# Autodesk Inventor assembly: endAssembly
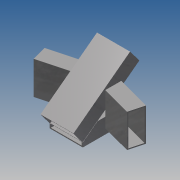
[picture p0: Inventor's stored thumbnail of the model, 180x180]
Saved by Autodesk Inventor 2013 SP2 (Build 170200200, 200)
## iProperties
Created: 2013-12-03
Part Number: endAssembly
Document SubType Name: Assembly
Designer: Dave
Author: Dave
## Documents named in this file (4)
- C:\Users\Dave\Desktop\hera-cad\support\endAssembly.iam
- C:\Users\Dave\Desktop\hera-cad\support\endHoriz.ipt
- C:\Users\Dave\Desktop\hera-cad\support\end37.ipt
- C:\Users\Dave\Desktop\hera-cad\support\endVert.ipt
## Components (4 placed, 3 different names)
1. endHoriz:1 — Mate:1, Mate:2, Mate:3
2. end37:1 — Mate:1
3. endVert:1 — Mate:3
4. endVert:2 — Mate:2
## Relationships (3: Mate 3)
- Mate:1: endHoriz:1 ↔ end37:1
- Mate:2: endHoriz:1 ↔ endVert:2
- Mate:3: endHoriz:1 ↔ endVert:1
